# Autodesk Inventor assembly: Assembly2
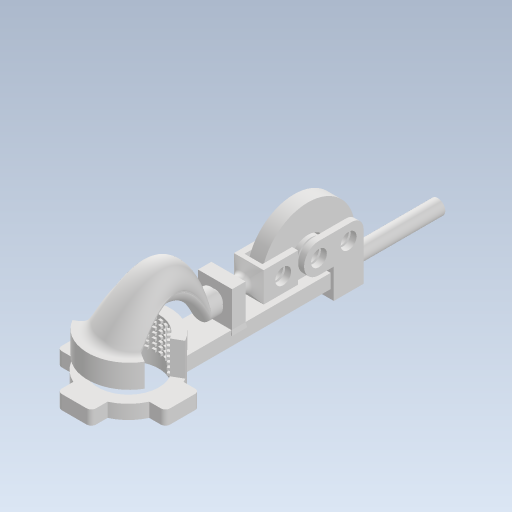
[picture p0: Inventor's stored thumbnail of the model, 512x512]
Saved by Autodesk Inventor 2023 (Build 270158000, 158)
## iProperties
Created: 2022-09-15
Part Number: Assembly2
Document SubType Name: Assembly
Designer: Dave
Author: Dave
## Documents named in this file (8)
- C:\Users\Dave\Desktop\Assembly2.iam
- C:\Users\Dave\Desktop\Plunger Cap.ipt
- C:\Users\Dave\Desktop\Plunger.ipt
- C:\Users\Dave\Desktop\Slider2.ipt
- C:\Users\Dave\Desktop\Support Hole.ipt
- C:\Users\Dave\Desktop\Locker.ipt
- C:\Users\Dave\Desktop\Tensioner2.ipt
- C:\Users\Dave\Desktop\Lever Arm.ipt
## Components (7 placed, 7 different names)
1. Plunger Cap:1 — Angle:2, Insert:1
2. Plunger:1 — Mate:3, Angle:1, Mate:8, Mate:10, Insert:1
3. Slider2:1 — Mate:1, Flush:1, Mate:2, Angle:1, Mate:6, Mate:7, Angle:2, Angle:3
4. Support Hole:1 — Mate:1, Flush:1, Mate:2, Mate:3
5. Locker:1 — Mate:6, Mate:7, Mate:9, Angle:3, Insert:2
6. Tensioner2:1 — Mate:8, Mate:9, Mate:10
7. Lever Arm:1 — Insert:2
## Relationships (14: Mate 8, Angle 3, Insert 2, Flush 1)
- Mate:1: Slider2:1 ↔ Support Hole:1
- Flush:1: Slider2:1 ↔ Support Hole:1
- Mate:2: Slider2:1 ↔ Support Hole:1
- Mate:3: Plunger:1 ↔ Support Hole:1
- Angle:1 (0 deg): Plunger:1 ↔ Slider2:1
- Mate:6: Slider2:1 ↔ Locker:1
- Mate:7 (0.801 mm): Slider2:1 ↔ Locker:1
- Mate:8: Plunger:1 ↔ Tensioner2:1
- Mate:9: Locker:1 ↔ Tensioner2:1
- Mate:10 (0.802 mm): Plunger:1 ↔ Tensioner2:1
- Angle:2 (0 deg): Plunger Cap:1 ↔ Slider2:1
- Insert:1: Plunger Cap:1 ↔ Plunger:1
- Angle:3 (-90 deg): Slider2:1 ↔ Locker:1
- Insert:2: Locker:1 ↔ Lever Arm:1
